# Autodesk Inventor assembly: shuttle cock assembly 2
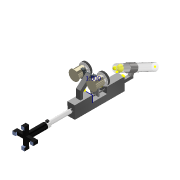
[picture p0: Inventor's stored thumbnail of the model, 180x180]
Saved by Autodesk Inventor 2021 (Build 250183000, 183)
## iProperties
Created: 2021-07-01
Part Number: shuttle cock assembly 2
Document SubType Name: Assembly
Designer: user
Author: user
## Documents named in this file (11)
- C:\Users\user\Desktop\New folder\shuttle cock assembly 2.iam
- C:\Users\user\Desktop\New folder\exploration cuboid.ipt
- C:\Users\user\Desktop\New folder\dc motor 2.ipt
- C:\Users\user\Desktop\New folder\cock clamp.ipt
- C:\Users\user\Desktop\New folder\cock storage.ipt
- C:\Users\user\Desktop\New folder\cock storage holder.ipt
- C:\Users\user\Desktop\New folder\stand.ipt
- C:\Users\user\Desktop\New folder\dc motor holder 2.ipt
- C:\Users\user\Desktop\New folder\cock wheel.ipt
- C:\Users\user\Desktop\New folder\Gripping Claws.ipt
- C:\Users\user\Desktop\New folder\cock1.ipt
## Components (13 placed, 10 different names)
1. exploration cuboid:1 — Mate:1, Mate:2, Mate:3, Mate:6, Mate:7, Mate:8, Mate:13, Mate:14, Mate:16, Mate:17
2. dc motor 2:1 — Mate:9, Flush:3, Mate:12, Flush:6, Rotational:1
3. dc motor 2:2 — Mate:10, Flush:4, Mate:11, Flush:5
4. cock clamp:1 — Mate:5, Flush:2
5. cock clamp:2 — Mate:4, Flush:1
6. cock storage:1 — Mate:15, Mate:18
7. cock storage holder:1 — Mate:13, Mate:14, Mate:15
8. stand:1 — Mate:1, Mate:2
9. dc motor holder 2:1 — Mate:6, Mate:7, Mate:8, Mate:9, Flush:3, Mate:10, Flush:4
10. cock wheel:1 — Mate:11, Flush:5
11. cock wheel:2 — Mate:12, Flush:6, Rotational:1
12. Gripping Claws:1 — Mate:3, Mate:4, Flush:1, Mate:5, Flush:2, Mate:16, Mate:17
13. cock1:1 — Mate:18
## Relationships (25: Mate 18, Flush 6, RevoluteJoint 1)
- Mate:1: exploration cuboid:1 ↔ stand:1
- Mate:2: exploration cuboid:1 ↔ stand:1
- Mate:3: exploration cuboid:1 ↔ Gripping Claws:1
- Mate:4: cock clamp:2 ↔ Gripping Claws:1
- Flush:1: cock clamp:2 ↔ Gripping Claws:1
- Mate:5: cock clamp:1 ↔ Gripping Claws:1
- Flush:2: cock clamp:1 ↔ Gripping Claws:1
- Mate:6: exploration cuboid:1 ↔ dc motor holder 2:1
- Mate:7: exploration cuboid:1 ↔ dc motor holder 2:1
- Mate:8 (53.34 mm): exploration cuboid:1 ↔ dc motor holder 2:1
- Mate:9: dc motor 2:1 ↔ dc motor holder 2:1
- Flush:3 (-19.05 mm): dc motor 2:1 ↔ dc motor holder 2:1
- Mate:10: dc motor 2:2 ↔ dc motor holder 2:1
- Flush:4 (-19.05 mm): dc motor 2:2 ↔ dc motor holder 2:1
- Mate:11: dc motor 2:2 ↔ cock wheel:1
- Flush:5 (-6.35 mm): dc motor 2:2 ↔ cock wheel:1
- Mate:12: dc motor 2:1 ↔ cock wheel:2
- Flush:6 (-6.35 mm): dc motor 2:1 ↔ cock wheel:2
- Mate:13: exploration cuboid:1 ↔ cock storage holder:1
- Mate:14: exploration cuboid:1 ↔ cock storage holder:1
- Mate:15: cock storage:1 ↔ cock storage holder:1
- Rotational:1 [RevoluteJoint] (-6.35 mm): dc motor 2:1 ↔ cock wheel:2
- Mate:16: exploration cuboid:1 ↔ Gripping Claws:1
- Mate:17: exploration cuboid:1 ↔ Gripping Claws:1
- Mate:18: cock storage:1 ↔ cock1:1
